# Autodesk Inventor assembly: Trunk
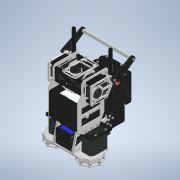
[picture p0: Inventor's stored thumbnail of the model, 180x180]
Saved by Autodesk Inventor 2020.4 (Build 244396000, 396)
## iProperties
Created: 2021-09-10
Part Number: Trunk
Document SubType Name: Assembly
Designer: Masato
Mass: 1616.91 g
Surface Area: 5782.28 cm^2
Volume: 882.028 cm^3
Density: 1.83317 g/cm^3
Author: Masato
## Documents named in this file (36)
- C:\Users\Masato\Documents\Inventor\CIT Brains_Inventor\OpenPlatform_ver3_0（ワッシャ変更）\UpperBody\Trunk\Trunk.iam
- C:\Users\Masato\Documents\Inventor\CIT Brains_Inventor\OpenPlatform_ver3_0（ワッシャ変更）\UpperBody\Trunk\Trunk_chest_horizontal_frame.ipt
- C:\Users\Masato\Documents\Inventor\CIT Brains_Inventor\OpenPlatform_ver3_0（ワッシャ変更）\UpperBody\Trunk\Trunk_chest_back_forth_frame.ipt
- C:\Users\Masato\Documents\Inventor\CIT Brains_Inventor\OpenPlatform_ver3_0（ワッシャ変更）\UpperBody\Trunk\Trunk_armpit_frame.ipt
- C:\Users\Masato\Documents\Inventor\CIT Brains_Inventor\OpenPlatform_ver3_0（ワッシャ変更）\UpperBody\Trunk\Trunk_abdomen_spacer.ipt
- C:\Users\Masato\Documents\Inventor\CIT Brains_Inventor\OpenPlatform_ver3_0（ワッシャ変更）\UpperBody\Trunk\Trunk_upper_flank_frame.ipt
- C:\Users\Masato\Documents\Inventor\CIT Brains_Inventor\OpenPlatform_ver3_0（ワッシャ変更）\UpperBody\Trunk\Trunk_shoulder_frame.ipt
- C:\Users\Masato\Documents\Inventor\CIT Brains_Inventor\OpenPlatform_ver3_0（ワッシャ変更）\UpperBody\Trunk\Trunk_handle_frame.ipt
- C:\Users\Masato\Documents\Inventor\CIT Brains_Inventor\OpenPlatform_ver3_0（ワッシャ変更）\UpperBody\Trunk\Trunk_chest_side_frame.ipt
- C:\Users\Masato\Documents\Inventor\CIT Brains_Inventor\OpenPlatform_ver3_0（ワッシャ変更）\Ready_Made\B3M11xx.ipt
- C:\Users\Masato\Documents\Inventor\CIT Brains_Inventor\OpenPlatform_ver3_0（ワッシャ変更）\Ready_Made\S3-07-3W.ipt
- C:\Users\Masato\Documents\Inventor\CIT Brains_Inventor\OpenPlatform_ver3_0（ワッシャ変更）\Ready_Made\ASU-375H.ipt
- C:\Users\Masato\Documents\Inventor\CIT Brains_Inventor\OpenPlatform_ver3_0（ワッシャ変更）\Ready_Made\B3M10xx.ipt
- C:\Users\Masato\Documents\Inventor\CIT Brains_Inventor\OpenPlatform_ver3_0（ワッシャ変更）\UpperBody\Cockpit\Cockpit.iam
- C:\Users\Masato\Documents\Inventor\CIT Brains_Inventor\OpenPlatform_ver3_0（ワッシャ変更）\UpperBody\Trunk\Trunk_shoulder_frame_MIR.ipt
- C:\Users\Masato\Documents\Inventor\CIT Brains_Inventor\OpenPlatform_ver3_0（ワッシャ変更）\UpperBody\Trunk\Trunk_lower_flank_frame.ipt
- C:\Users\Masato\Documents\Inventor\CIT Brains_Inventor\OpenPlatform_ver3_0（ワッシャ変更）\Ready_Made\Screw\SPNFL-BRN-M3-6.ipt
- C:\Users\Masato\Documents\Inventor\CIT Brains_Inventor\OpenPlatform_ver3_0（ワッシャ変更）\Ready_Made\Screw\M2_6-15.ipt
- C:\Users\Masato\Documents\Inventor\CIT Brains_Inventor\OpenPlatform_ver3_0（ワッシャ変更）\Ready_Made\Screw\M3-8.ipt
- C:\Users\Masato\Documents\Inventor\CIT Brains_Inventor\OpenPlatform_ver3_0（ワッシャ変更）\Ready_Made\Screw\M3-6.ipt
- C:\Users\Masato\Documents\Inventor\CIT Brains_Inventor\OpenPlatform_ver3_0（ワッシャ変更）\Ready_Made\Screw\M2_6-20.ipt
- C:\Users\Masato\Documents\Inventor\CIT Brains_Inventor\OpenPlatform_ver3_0（ワッシャ変更）\UpperBody\Trunk\Outer_support_stand.ipt
- C:\Users\Masato\Documents\Inventor\CIT Brains_Inventor\OpenPlatform_ver3_0（ワッシャ変更）\Ready_Made\BRU-307S.ipt
- C:\Users\Masato\Documents\Inventor\CIT Brains_Inventor\OpenPlatform_ver3_0（ワッシャ変更）\UpperBody\Trunk\Outer_flange.ipt
- C:\Users\Masato\Documents\Inventor\CIT Brains_Inventor\OpenPlatform_ver3_0（ワッシャ変更）\UpperBody\Trunk\Inner_flange.ipt
- C:\Users\Masato\Documents\Inventor\CIT Brains_Inventor\OpenPlatform_ver3_0（ワッシャ変更）\Ready_Made\CRBA02508WWC8P5\CRBA02508WWC8P5.ipt
- C:\Users\Masato\Documents\Inventor\CIT Brains_Inventor\OpenPlatform_ver3_0（ワッシャ変更）\UpperBody\Trunk\Inner_support_stand.ipt
- C:\Users\Masato\Documents\Inventor\CIT Brains_Inventor\OpenPlatform_ver3_0（ワッシャ変更）\UpperBody\Trunk\Trunk_lower_waisit_frame.ipt
- C:\Users\Masato\Documents\Inventor\CIT Brains_Inventor\OpenPlatform_ver3_0（ワッシャ変更）\Ready_Made\BRU-309S.ipt
- C:\Users\Masato\Documents\Inventor\CIT Brains_Inventor\OpenPlatform_ver3_0（ワッシャ変更）\UpperBody\Trunk\Trunk_upper_waist_frame.ipt
- C:\Users\Masato\Documents\Inventor\CIT Brains_Inventor\OpenPlatform_ver3_0（ワッシャ変更）\Ready_Made\UUW-0312-10BH.ipt
- C:\Users\Masato\Documents\Inventor\CIT Brains_Inventor\OpenPlatform_ver3_0（ワッシャ変更）\Ready_Made\Screw\M2_6-6.ipt
- C:\Users\Masato\Documents\Inventor\CIT Brains_Inventor\OpenPlatform_ver3_0（ワッシャ変更）\Ready_Made\ASU-309-6.ipt
- C:\Users\Masato\Documents\Inventor\CIT Brains_Inventor\OpenPlatform_ver3_0（ワッシャ変更）\Ready_Made\SLSBF7-134-M3-N3.ipt
- C:\Users\Masato\Documents\Inventor\CIT Brains_Inventor\OpenPlatform_ver3_0（ワッシャ変更）\Ready_Made\BRU-2608S.ipt
- C:\Users\Masato\Documents\Inventor\CIT Brains_Inventor\OpenPlatform_ver3_0（ワッシャ変更）\Ready_Made\SF319.ipt
## Components (214 placed, 35 different names)
1. Trunk_chest_horizontal_frame:1 — 挿入:172, 挿入:173, 挿入:174, 挿入:175, 挿入:177, 挿入:179, 挿入:255, 挿入:256, 挿入:261, 挿入:262, 挿入:347, 挿入:348, 挿入:463, 挿入:464
2. Trunk_chest_horizontal_frame:2 — 挿入:181, 挿入:182, 挿入:184, 挿入:185, 挿入:186, 挿入:187, 挿入:257, 挿入:258, 挿入:337, 挿入:338, 挿入:465, 挿入:466, 挿入:664, 挿入:665
3. Trunk_chest_back_forth_frame:1 — 挿入:115, 挿入:116, 挿入:117, 挿入:118, 挿入:172, 挿入:173, 挿入:181, 挿入:182
4. Trunk_chest_back_forth_frame:2 — 挿入:154, 挿入:155, 挿入:156, 挿入:157, 挿入:174, 挿入:175, 挿入:185, 挿入:187
5. Trunk_armpit_frame:1 — 挿入:111, 挿入:112, 挿入:555, 挿入:556
6. Trunk_armpit_frame:2 — 挿入:164, 挿入:165, 挿入:557, 挿入:558
7. Trunk_armpit_frame:3 — 挿入:229, 挿入:230, 挿入:577, 挿入:579
8. Trunk_armpit_frame:4 — 挿入:168, 挿入:169, 挿入:578, 挿入:580
9. Trunk_lower_flank_frame:1 — 挿入:420, 挿入:421, 挿入:426, 挿入:501, 挿入:502, 挿入:668, 挿入:669
10. Trunk_lower_flank_frame:2 — メイト:23, メイト:24, メイト:25, 挿入:418, 挿入:419, 挿入:499, 挿入:500, 挿入:666, 挿入:667
11. Trunk_abdomen_spacer:1 — フラッシュ:16, メイト:17, フラッシュ:18, フラッシュ:20, フラッシュ:21, メイト:22
12. Trunk_abdomen_spacer:2 — フラッシュ:16, メイト:17, フラッシュ:18, メイト:19
13. Trunk_abdomen_spacer:3 — フラッシュ:15, メイト:18, フラッシュ:17, フラッシュ:19, フラッシュ:20, フラッシュ:21, メイト:21, メイト:20
14. Trunk_abdomen_spacer:4 — フラッシュ:15, メイト:18, フラッシュ:17, メイト:25
15. Trunk_upper_flank_frame:1 — 挿入:101, 挿入:102, 挿入:103, 挿入:111, 挿入:112, 挿入:115, 挿入:116, 挿入:156, 挿入:157, 挿入:164, 挿入:165, フラッシュ:19, メイト:21, 挿入:208, 挿入:226, 挿入:245, 挿入:246, 挿入:247, 挿入:251, 挿入:252, 挿入:327, 挿入:328, 挿入:329, 挿入:330, 挿入:349, 挿入:350
16. Trunk_upper_flank_frame:2 — 挿入:104, 挿入:105, 挿入:106, 挿入:117, 挿入:118, 挿入:154, 挿入:155, 挿入:168, 挿入:169, メイト:22, 挿入:227, 挿入:229, 挿入:230, 挿入:248, 挿入:249, 挿入:250, 挿入:253, 挿入:254, 挿入:331, 挿入:332, 挿入:333, 挿入:334, 挿入:351, 挿入:352
17. Trunk_shoulder_frame:1 — 挿入:555, 挿入:556, 挿入:557, 挿入:558, 挿入:559, 挿入:560, 挿入:561, 挿入:562, 挿入:563, 挿入:564, 挿入:565, 挿入:566, 挿入:567, 挿入:568, 挿入:569, 挿入:570, 角度:48, 挿入:571, 角度:49, 挿入:572, 挿入:573, 挿入:574
18. Trunk_shoulder_frame_MIR:1 — 挿入:577, 挿入:578, 挿入:579, 挿入:580, 挿入:581, 挿入:582, 挿入:583, 挿入:584, 挿入:585, 挿入:586, 挿入:587, 挿入:588, 挿入:589, 挿入:590, 挿入:591, 挿入:592, 挿入:593, 挿入:594, 角度:50, 角度:51, 挿入:595, 挿入:596
19. Trunk_handle_frame:1 — 挿入:263, 挿入:264, 挿入:267, 挿入:575, 挿入:576, 角度:52, 挿入:599
20. Trunk_handle_frame:2 — 挿入:265, 挿入:266, 挿入:268, 挿入:597, 挿入:598
21. Trunk_chest_side_frame:1 — 挿入:467, 挿入:468, 挿入:469, 挿入:470, 挿入:471, 挿入:472, 挿入:473, 挿入:474
22. Trunk_chest_side_frame:2 — 挿入:475, 挿入:476, 挿入:477, 挿入:478, 挿入:479, 挿入:480, 挿入:481, 挿入:482
23. B3M11xx:1 — 角度:39, 挿入:391, 挿入:392, 挿入:422, 挿入:423, 挿入:424, 挿入:425, 挿入:483, 挿入:486, フラッシュ:23
24. B3M11xx:2 — 挿入:427, 挿入:428, 挿入:429, 挿入:484, 挿入:485, 挿入:529
25. B3M11xx:3 — 挿入:177, 挿入:179, 挿入:184, 挿入:186
26. B3M10xx:4 — 挿入:475, 挿入:476, 挿入:477, 挿入:478, 挿入:559, 挿入:560, 挿入:561, 挿入:562
27. B3M10xx:5 — 挿入:467, 挿入:468, 挿入:469, 挿入:470, 挿入:581, 挿入:582, 挿入:583, 挿入:584
28. ASU-375H:1 — フラッシュ:9, フラッシュ:10, フラッシュ:11, フラッシュ:12, 挿入:101, 挿入:104, メイト:19, メイト:20, メイト:23, メイト:24
29. ASU-375H:2 — フラッシュ:9, フラッシュ:11, 挿入:102, 挿入:105
30. ASU-375H:3 — フラッシュ:10, フラッシュ:12, 挿入:103, 挿入:106
31. Cockpit:1 [sub-assembly] — 挿入:208, 角度:39
32. SPNFL-BRN-M3-6:1 — 挿入:226
33. SPNFL-BRN-M3-6:2 — 挿入:227
34. M3-8:5 — 挿入:245
35. M3-8:6 — 挿入:246
36. M3-8:7 — 挿入:247
37. M3-8:8 — 挿入:248
38. M3-8:9 — 挿入:249
39. M3-8:10 — 挿入:250
40. M3-6:1 — 挿入:251
41. M3-6:2 — 挿入:252
42. M3-6:3 — 挿入:254
43. M3-6:4 — 挿入:253
44. M3-6:5 — 挿入:256
45. M3-6:6 — 挿入:255
46. M3-6:7 — 挿入:258
47. M3-6:8 — 挿入:257
48. M2_6-15:9 — 挿入:464
49. M2_6-15:10 — 挿入:463
50. M2_6-15:11 — 挿入:261
51. M2_6-15:12 — 挿入:262
52. M3-6:9 — 挿入:263
53. M3-6:10 — 挿入:264
54. M3-6:11 — 挿入:266
55. M3-6:12 — 挿入:265
56. M3-8:11 — 挿入:267
57. M3-8:12 — 挿入:268
58. M2_6-20:1 — 挿入:489
59. M2_6-20:2 — 挿入:490
60. M2_6-20:3 — 挿入:487
61. M2_6-20:4 — 挿入:488
62. M2_6-15:13 — 挿入:564
63. M2_6-15:14 — 挿入:563
64. M2_6-15:15 — 挿入:566
65. M2_6-15:16 — 挿入:565
66. M2_6-15:17 — 挿入:591
67. M2_6-15:18 — 挿入:592
68. M2_6-15:19 — 挿入:589
69. M2_6-15:20 — 挿入:590
70. M3-6:13 — 挿入:567
71. M3-6:14 — 挿入:568
72. M3-6:15 — 挿入:569
73. M3-6:16 — 挿入:570
74. M3-6:17 — 挿入:585
75. M3-6:18 — 挿入:586
76. M3-6:19 — 挿入:587
77. M3-6:20 — 挿入:588
78. M3-6:21 — 挿入:327
79. M3-6:22 — 挿入:328
80. M3-6:23 — 挿入:329
81. M3-6:24 — 挿入:330
82. M3-6:25 — 挿入:331
83. M3-6:26 — 挿入:332
84. M3-6:27 — 挿入:333
85. M3-6:28 — 挿入:334
86. M2_6-20:9 — 挿入:465
87. M2_6-20:10 — 挿入:466
88. M2_6-20:11 — 挿入:337
89. M2_6-20:12 — 挿入:338
90. M2_6-20:13 — 挿入:479
91. M2_6-20:14 — 挿入:482
92. M2_6-20:15 — 挿入:481
93. M2_6-20:16 — 挿入:480
94. M2_6-20:17 — 挿入:474
95. M2_6-20:18 — 挿入:472
96. M2_6-20:19 — 挿入:473
97. M2_6-20:20 — 挿入:471
98. M3-6:29 — 挿入:347
99. M3-6:30 — 挿入:348
100. M3-6:31 — 挿入:349
101. M3-6:32 — 挿入:350
102. M3-6:33 — 挿入:351
103. M3-6:34 — 挿入:352
104. Outer_support_stand:1 — 挿入:397, 挿入:600, 挿入:601, 挿入:602, 挿入:603, 挿入:604, 挿入:605, 挿入:606, 挿入:607, 挿入:608, 挿入:609
105. Inner_flange:1 — 挿入:391, 挿入:392, 挿入:652, 挿入:653, 挿入:654, 挿入:655
106. CRBA02508WWC8P5:1 — 挿入:397
107. Inner_support_stand:1 — 角度:53, 角度:54, 角度:55, 角度:56, 挿入:624, 挿入:625, 挿入:626, 挿入:627, 挿入:644, 挿入:645, 挿入:646, 挿入:647, 挿入:662, 挿入:663
108. S3-07-3W:9 — 角度:53, 挿入:625
109. S3-07-3W:10 — 角度:56, 挿入:626
110. S3-07-3W:11 — 角度:55, 挿入:627
111. S3-07-3W:12 — 角度:54, 挿入:624
112. Outer_flange:1 — 挿入:406, 挿入:407, 挿入:408, 挿入:409, 挿入:410, 挿入:411, 挿入:412, 挿入:413, 挿入:610, 挿入:611
113. M3-6:35 — 挿入:406
114. M3-6:36 — 挿入:407
115. M3-6:37 — 挿入:408
116. M3-6:38 — 挿入:409
117. M3-6:39 — 挿入:410
118. M3-6:40 — 挿入:411
119. M3-6:41 — 挿入:412
120. M3-6:42 — 挿入:413
121. Trunk_lower_waisit_frame:1 — 挿入:418, 挿入:419, 挿入:420, 挿入:421, 挿入:422, 挿入:423, 挿入:424, 挿入:425, 挿入:426, 挿入:427, 挿入:428, 挿入:429, 挿入:440, 挿入:441, 挿入:442, 挿入:443, 挿入:444, 挿入:445, 挿入:446, 挿入:447, 挿入:448, 挿入:449, 挿入:450, 挿入:451, フラッシュ:22, 挿入:600, 挿入:601, 挿入:612, 挿入:623
122. M2_6-15:21 — 挿入:441
123. M2_6-15:22 — 挿入:440
124. M2_6-15:23 — 挿入:442
125. M2_6-15:24 — 挿入:443
126. M2_6-15:25 — 挿入:444
127. M2_6-15:26 — 挿入:445
128. M2_6-15:27 — 挿入:446
129. M2_6-15:28 — 挿入:447
130. M3-8:13 — 挿入:448
131. M3-8:14 — 挿入:449
132. M3-8:15 — 挿入:450
133. M3-8:16 — 挿入:451
134. Trunk_upper_waist_frame:1 — 挿入:483, 挿入:484, 挿入:485, 挿入:486, 挿入:487, 挿入:488, 挿入:489, 挿入:490
135. BRU-307S:9 — 挿入:497, 挿入:503
136. BRU-307S:10 — 挿入:498, 挿入:504
137. BRU-307S:11 — 挿入:496, 挿入:506
138. BRU-307S:12 — 挿入:495, 挿入:505
139. UUW-0312-10BH:1 — 挿入:495, 挿入:507
140. UUW-0312-10BH:2 — 挿入:496, 挿入:508
141. UUW-0312-10BH:3 — 挿入:497, 挿入:509
142. UUW-0312-10BH:4 — 挿入:498, 挿入:510
143. UUW-0312-10BH:5 — 挿入:499, 挿入:505
144. UUW-0312-10BH:6 — 挿入:500, 挿入:506
145. UUW-0312-10BH:7 — 挿入:501, 挿入:503
146. UUW-0312-10BH:8 — 挿入:502, 挿入:504
147. M3-6:43 — 挿入:507
148. M3-6:44 — 挿入:508
149. M3-6:45 — 挿入:510
150. M3-6:46 — 挿入:509
151. Outer_support_stand:2 — 挿入:554, 挿入:612, 挿入:613, 挿入:614, 挿入:615, 挿入:616, 挿入:617, 挿入:618, 挿入:619, 挿入:620, 挿入:623
152. S3-07-3W:13 — 角度:59, 挿入:630
153. S3-07-3W:14 — 角度:58, 挿入:629
154. S3-07-3W:15 — 角度:60, 挿入:631
155. S3-07-3W:16 — 角度:57, 挿入:628
156. Inner_flange:2 — 挿入:529, 挿入:656, 挿入:657, 挿入:658, 挿入:659
157. Inner_support_stand:2 — 角度:57, 角度:58, 角度:59, 角度:60, 挿入:628, 挿入:629, 挿入:630, 挿入:631, 挿入:648, 挿入:649, 挿入:650, 挿入:651, 挿入:660, 挿入:661
158. Outer_flange:2 — 挿入:542, 挿入:543, 挿入:544, 挿入:545, 挿入:546, 挿入:547, 挿入:548, 挿入:549, 挿入:621, 挿入:622
159. M3-6:47 — 挿入:542
160. M3-6:48 — 挿入:543
161. M3-6:49 — 挿入:544
162. M3-6:50 — 挿入:545
163. M3-6:51 — 挿入:546
164. M3-6:52 — 挿入:547
165. M3-6:53 — 挿入:548
166. M3-6:54 — 挿入:549
167. CRBA02508WWC8P5:2 — 挿入:554
168. ASU-309-6:1 — 角度:48, 挿入:571, 挿入:576
169. ASU-309-6:2 — 角度:49, 挿入:572, 挿入:575
170. M3-6:55 — 挿入:573
171. M3-6:56 — 挿入:574
172. M3-6:57 — 挿入:593
173. M3-6:58 — 挿入:594
174. ASU-309-6:3 — 角度:50, 挿入:595, 挿入:597
175. ASU-309-6:4 — 角度:51, 挿入:596, 挿入:598
176. SLSBF7-134-M3-N3:1 — 角度:52, 挿入:599
177. BRU-309S:17 — 挿入:602, 挿入:610
178. BRU-309S:18 — 挿入:603
179. BRU-309S:19 — 挿入:604
180. BRU-309S:20 — 挿入:605
181. BRU-309S:21 — 挿入:606, 挿入:611
182. BRU-309S:22 — 挿入:607
183. BRU-309S:23 — 挿入:608
184. BRU-309S:24 — 挿入:609
185. BRU-309S:25 — 挿入:617
186. BRU-309S:26 — 挿入:616
187. BRU-309S:27 — 挿入:615
188. BRU-309S:28 — 挿入:613, 挿入:621
189. BRU-309S:29 — 挿入:614
190. BRU-309S:30 — 挿入:618
191. BRU-309S:31 — 挿入:619
192. BRU-309S:32 — 挿入:620, 挿入:622
193. M2_6-6:1 — 挿入:644
194. M2_6-6:2 — 挿入:645
195. M2_6-6:3 — 挿入:646
196. M2_6-6:4 — 挿入:647
197. M2_6-6:5 — 挿入:651
198. M2_6-6:6 — 挿入:650
199. M2_6-6:7 — 挿入:649
200. M2_6-6:8 — 挿入:648
201. BRU-2608S:1 — 挿入:653, 挿入:662
202. BRU-2608S:2 — 挿入:654, 挿入:663
203. BRU-2608S:3 — 挿入:655
204. BRU-2608S:4 — 挿入:652
205. BRU-2608S:5 — 挿入:657, 挿入:660
206. BRU-2608S:6 — 挿入:656
207. BRU-2608S:7 — 挿入:658
208. BRU-2608S:8 — 挿入:659, 挿入:661
209. M3-6:59 — 挿入:664
210. M3-6:60 — 挿入:665
211. SF319:1 — 挿入:666
212. SF319:2 — 挿入:667
213. SF319:3 — 挿入:668
214. SF319:4 — 挿入:669
## Relationships (303: Insert 267, Angle 14, Flush 13, Mate 9)
- フラッシュ:9 [Flush]: ASU-375H:1 ↔ ASU-375H:2
- フラッシュ:10 [Flush]: ASU-375H:1 ↔ ASU-375H:3
- フラッシュ:11 [Flush]: ASU-375H:1 ↔ ASU-375H:2
- フラッシュ:12 [Flush]: ASU-375H:1 ↔ ASU-375H:3
- 挿入:101 [Insert]: Trunk_upper_flank_frame:1 ↔ ASU-375H:1
- 挿入:102 [Insert]: Trunk_upper_flank_frame:1 ↔ ASU-375H:2
- 挿入:103 [Insert]: Trunk_upper_flank_frame:1 ↔ ASU-375H:3
- 挿入:104 [Insert]: Trunk_upper_flank_frame:2 ↔ ASU-375H:1
- 挿入:105 [Insert]: Trunk_upper_flank_frame:2 ↔ ASU-375H:2
- 挿入:106 [Insert]: Trunk_upper_flank_frame:2 ↔ ASU-375H:3
- 挿入:111 [Insert]: Trunk_armpit_frame:1 ↔ Trunk_upper_flank_frame:1
- 挿入:112 [Insert]: Trunk_armpit_frame:1 ↔ Trunk_upper_flank_frame:1
- 挿入:115 [Insert]: Trunk_chest_back_forth_frame:1 ↔ Trunk_upper_flank_frame:1
- 挿入:116 [Insert]: Trunk_chest_back_forth_frame:1 ↔ Trunk_upper_flank_frame:1
- 挿入:117 [Insert]: Trunk_chest_back_forth_frame:1 ↔ Trunk_upper_flank_frame:2
- 挿入:118 [Insert]: Trunk_chest_back_forth_frame:1 ↔ Trunk_upper_flank_frame:2
- 挿入:154 [Insert]: Trunk_chest_back_forth_frame:2 ↔ Trunk_upper_flank_frame:2
- 挿入:155 [Insert]: Trunk_chest_back_forth_frame:2 ↔ Trunk_upper_flank_frame:2
- 挿入:156 [Insert]: Trunk_chest_back_forth_frame:2 ↔ Trunk_upper_flank_frame:1
- 挿入:157 [Insert]: Trunk_chest_back_forth_frame:2 ↔ Trunk_upper_flank_frame:1
- 挿入:164 [Insert]: Trunk_armpit_frame:2 ↔ Trunk_upper_flank_frame:1
- 挿入:165 [Insert]: Trunk_armpit_frame:2 ↔ Trunk_upper_flank_frame:1
- 挿入:168 [Insert]: Trunk_armpit_frame:4 ↔ Trunk_upper_flank_frame:2
- 挿入:169 [Insert]: Trunk_armpit_frame:4 ↔ Trunk_upper_flank_frame:2
- 挿入:172 [Insert]: Trunk_chest_horizontal_frame:1 ↔ Trunk_chest_back_forth_frame:1
- 挿入:173 [Insert]: Trunk_chest_horizontal_frame:1 ↔ Trunk_chest_back_forth_frame:1
- 挿入:174 [Insert]: Trunk_chest_horizontal_frame:1 ↔ Trunk_chest_back_forth_frame:2
- 挿入:175 [Insert]: Trunk_chest_horizontal_frame:1 ↔ Trunk_chest_back_forth_frame:2
- 挿入:177 [Insert]: Trunk_chest_horizontal_frame:1 ↔ B3M11xx:3
- 挿入:179 [Insert]: Trunk_chest_horizontal_frame:1 ↔ B3M11xx:3
- 挿入:181 [Insert]: Trunk_chest_horizontal_frame:2 ↔ Trunk_chest_back_forth_frame:1
- 挿入:182 [Insert]: Trunk_chest_horizontal_frame:2 ↔ Trunk_chest_back_forth_frame:1
- 挿入:184 [Insert]: Trunk_chest_horizontal_frame:2 ↔ B3M11xx:3
- 挿入:185 [Insert]: Trunk_chest_horizontal_frame:2 ↔ Trunk_chest_back_forth_frame:2
- 挿入:186 [Insert]: Trunk_chest_horizontal_frame:2 ↔ B3M11xx:3
- 挿入:187 [Insert]: Trunk_chest_horizontal_frame:2 ↔ Trunk_chest_back_forth_frame:2
- フラッシュ:15 [Flush]: Trunk_abdomen_spacer:3 ↔ Trunk_abdomen_spacer:4
- フラッシュ:16 [Flush]: Trunk_abdomen_spacer:1 ↔ Trunk_abdomen_spacer:2
- メイト:17 [Mate]: Trunk_abdomen_spacer:1 ↔ Trunk_abdomen_spacer:2
- メイト:18 [Mate]: Trunk_abdomen_spacer:3 ↔ Trunk_abdomen_spacer:4
- フラッシュ:17 [Flush]: Trunk_abdomen_spacer:3 ↔ Trunk_abdomen_spacer:4
- フラッシュ:18 [Flush]: Trunk_abdomen_spacer:1 ↔ Trunk_abdomen_spacer:2
- フラッシュ:19 [Flush]: Trunk_abdomen_spacer:3 ↔ Trunk_upper_flank_frame:1
- フラッシュ:20 [Flush]: Trunk_abdomen_spacer:1 ↔ Trunk_abdomen_spacer:3
- メイト:19 [Mate] (0.01 mm): Trunk_abdomen_spacer:2 ↔ ASU-375H:1
- メイト:20 [Mate] (0.01 mm): Trunk_abdomen_spacer:3 ↔ ASU-375H:1
- フラッシュ:21 [Flush]: Trunk_abdomen_spacer:1 ↔ Trunk_abdomen_spacer:3
- メイト:21 [Mate]: Trunk_abdomen_spacer:3 ↔ Trunk_upper_flank_frame:1
- メイト:22 [Mate]: Trunk_abdomen_spacer:1 ↔ Trunk_upper_flank_frame:2
- メイト:23 [Mate] (0.01 mm): Trunk_lower_flank_frame:2 ↔ ASU-375H:1
- メイト:24 [Mate] (0.01 mm): Trunk_lower_flank_frame:2 ↔ ASU-375H:1
- メイト:25 [Mate]: Trunk_lower_flank_frame:2 ↔ Trunk_abdomen_spacer:4
- 挿入:208 [Insert] (0.25 mm): Trunk_upper_flank_frame:1 ↔ Cockpit:1
- 角度:39 [Angle] (0 deg): B3M11xx:1 ↔ Cockpit:1
- 挿入:226 [Insert]: Trunk_upper_flank_frame:1 ↔ SPNFL-BRN-M3-6:1
- 挿入:227 [Insert]: Trunk_upper_flank_frame:2 ↔ SPNFL-BRN-M3-6:2
- 挿入:229 [Insert]: Trunk_armpit_frame:3 ↔ Trunk_upper_flank_frame:2
- 挿入:230 [Insert]: Trunk_armpit_frame:3 ↔ Trunk_upper_flank_frame:2
- 挿入:245 [Insert]: Trunk_upper_flank_frame:1 ↔ M3-8:5
- 挿入:246 [Insert]: Trunk_upper_flank_frame:1 ↔ M3-8:6
- 挿入:247 [Insert]: Trunk_upper_flank_frame:1 ↔ M3-8:7
- 挿入:248 [Insert]: Trunk_upper_flank_frame:2 ↔ M3-8:8
- 挿入:249 [Insert]: Trunk_upper_flank_frame:2 ↔ M3-8:9
- 挿入:250 [Insert]: Trunk_upper_flank_frame:2 ↔ M3-8:10
- 挿入:251 [Insert]: Trunk_upper_flank_frame:1 ↔ M3-6:1
- 挿入:252 [Insert]: Trunk_upper_flank_frame:1 ↔ M3-6:2
- 挿入:253 [Insert]: Trunk_upper_flank_frame:2 ↔ M3-6:4
- 挿入:254 [Insert]: Trunk_upper_flank_frame:2 ↔ M3-6:3
- 挿入:255 [Insert]: Trunk_chest_horizontal_frame:1 ↔ M3-6:6
- 挿入:256 [Insert]: Trunk_chest_horizontal_frame:1 ↔ M3-6:5
- 挿入:257 [Insert]: Trunk_chest_horizontal_frame:2 ↔ M3-6:8
- 挿入:258 [Insert]: Trunk_chest_horizontal_frame:2 ↔ M3-6:7
- 挿入:261 [Insert]: Trunk_chest_horizontal_frame:1 ↔ M2_6-15:11
- 挿入:262 [Insert]: Trunk_chest_horizontal_frame:1 ↔ M2_6-15:12
- 挿入:263 [Insert]: Trunk_handle_frame:1 ↔ M3-6:9
- 挿入:264 [Insert]: Trunk_handle_frame:1 ↔ M3-6:10
- 挿入:265 [Insert]: Trunk_handle_frame:2 ↔ M3-6:12
- 挿入:266 [Insert]: Trunk_handle_frame:2 ↔ M3-6:11
- 挿入:267 [Insert]: Trunk_handle_frame:1 ↔ M3-8:11
- 挿入:268 [Insert]: Trunk_handle_frame:2 ↔ M3-8:12
- 挿入:327 [Insert]: Trunk_upper_flank_frame:1 ↔ M3-6:21
- 挿入:328 [Insert]: Trunk_upper_flank_frame:1 ↔ M3-6:22
- 挿入:329 [Insert]: Trunk_upper_flank_frame:1 ↔ M3-6:23
- 挿入:330 [Insert]: Trunk_upper_flank_frame:1 ↔ M3-6:24
- 挿入:331 [Insert]: Trunk_upper_flank_frame:2 ↔ M3-6:25
- 挿入:332 [Insert]: Trunk_upper_flank_frame:2 ↔ M3-6:26
- 挿入:333 [Insert]: Trunk_upper_flank_frame:2 ↔ M3-6:27
- 挿入:334 [Insert]: Trunk_upper_flank_frame:2 ↔ M3-6:28
- 挿入:337 [Insert]: Trunk_chest_horizontal_frame:2 ↔ M2_6-20:11
- 挿入:338 [Insert]: Trunk_chest_horizontal_frame:2 ↔ M2_6-20:12
- 挿入:347 [Insert]: Trunk_chest_horizontal_frame:1 ↔ M3-6:29
- 挿入:348 [Insert]: Trunk_chest_horizontal_frame:1 ↔ M3-6:30
- 挿入:349 [Insert]: Trunk_upper_flank_frame:1 ↔ M3-6:31
- 挿入:350 [Insert]: Trunk_upper_flank_frame:1 ↔ M3-6:32
- 挿入:351 [Insert]: Trunk_upper_flank_frame:2 ↔ M3-6:33
- 挿入:352 [Insert]: Trunk_upper_flank_frame:2 ↔ M3-6:34
- 挿入:391 [Insert]: B3M11xx:1 ↔ Inner_flange:1
- 挿入:392 [Insert]: B3M11xx:1 ↔ Inner_flange:1
- 挿入:397 [Insert]: Outer_support_stand:1 ↔ CRBA02508WWC8P5:1
- 挿入:406 [Insert]: Outer_flange:1 ↔ M3-6:35
- 挿入:407 [Insert]: Outer_flange:1 ↔ M3-6:36
- 挿入:408 [Insert]: Outer_flange:1 ↔ M3-6:37
- 挿入:409 [Insert]: Outer_flange:1 ↔ M3-6:38
- 挿入:410 [Insert]: Outer_flange:1 ↔ M3-6:39
- 挿入:411 [Insert]: Outer_flange:1 ↔ M3-6:40
- 挿入:412 [Insert]: Outer_flange:1 ↔ M3-6:41
- 挿入:413 [Insert]: Outer_flange:1 ↔ M3-6:42
- 挿入:418 [Insert]: Trunk_lower_flank_frame:2 ↔ Trunk_lower_waisit_frame:1
- 挿入:419 [Insert]: Trunk_lower_flank_frame:2 ↔ Trunk_lower_waisit_frame:1
- 挿入:420 [Insert]: Trunk_lower_flank_frame:1 ↔ Trunk_lower_waisit_frame:1
- 挿入:421 [Insert]: Trunk_lower_flank_frame:1 ↔ Trunk_lower_waisit_frame:1
- 挿入:422 [Insert]: B3M11xx:1 ↔ Trunk_lower_waisit_frame:1
- 挿入:423 [Insert]: B3M11xx:1 ↔ Trunk_lower_waisit_frame:1
- 挿入:424 [Insert]: B3M11xx:1 ↔ Trunk_lower_waisit_frame:1
- 挿入:425 [Insert]: B3M11xx:1 ↔ Trunk_lower_waisit_frame:1
- 挿入:426 [Insert]: Trunk_lower_flank_frame:1 ↔ Trunk_lower_waisit_frame:1
- 挿入:427 [Insert]: B3M11xx:2 ↔ Trunk_lower_waisit_frame:1
- 挿入:428 [Insert]: B3M11xx:2 ↔ Trunk_lower_waisit_frame:1
- 挿入:429 [Insert]: B3M11xx:2 ↔ Trunk_lower_waisit_frame:1
- 挿入:440 [Insert]: Trunk_lower_waisit_frame:1 ↔ M2_6-15:22
- 挿入:441 [Insert]: Trunk_lower_waisit_frame:1 ↔ M2_6-15:21
- 挿入:442 [Insert]: Trunk_lower_waisit_frame:1 ↔ M2_6-15:23
- 挿入:443 [Insert]: Trunk_lower_waisit_frame:1 ↔ M2_6-15:24
- 挿入:444 [Insert]: Trunk_lower_waisit_frame:1 ↔ M2_6-15:25
- 挿入:445 [Insert]: Trunk_lower_waisit_frame:1 ↔ M2_6-15:26
- 挿入:446 [Insert]: Trunk_lower_waisit_frame:1 ↔ M2_6-15:27
- 挿入:447 [Insert]: Trunk_lower_waisit_frame:1 ↔ M2_6-15:28
- 挿入:448 [Insert]: Trunk_lower_waisit_frame:1 ↔ M3-8:13
- 挿入:449 [Insert]: Trunk_lower_waisit_frame:1 ↔ M3-8:14
- 挿入:450 [Insert]: Trunk_lower_waisit_frame:1 ↔ M3-8:15
- 挿入:451 [Insert]: Trunk_lower_waisit_frame:1 ↔ M3-8:16
- フラッシュ:22 [Flush]: Trunk_lower_waisit_frame:1
- 挿入:463 [Insert]: Trunk_chest_horizontal_frame:1 ↔ M2_6-15:10
- 挿入:464 [Insert]: Trunk_chest_horizontal_frame:1 ↔ M2_6-15:9
- 挿入:465 [Insert]: Trunk_chest_horizontal_frame:2 ↔ M2_6-20:9
- 挿入:466 [Insert]: Trunk_chest_horizontal_frame:2 ↔ M2_6-20:10
- 挿入:467 [Insert]: Trunk_chest_side_frame:1 ↔ B3M10xx:5
- 挿入:468 [Insert]: Trunk_chest_side_frame:1 ↔ B3M10xx:5
- 挿入:469 [Insert]: Trunk_chest_side_frame:1 ↔ B3M10xx:5
- 挿入:470 [Insert]: Trunk_chest_side_frame:1 ↔ B3M10xx:5
- 挿入:471 [Insert]: Trunk_chest_side_frame:1 ↔ M2_6-20:20
- 挿入:472 [Insert]: Trunk_chest_side_frame:1 ↔ M2_6-20:18
- 挿入:473 [Insert]: Trunk_chest_side_frame:1 ↔ M2_6-20:19
- 挿入:474 [Insert]: Trunk_chest_side_frame:1 ↔ M2_6-20:17
- 挿入:475 [Insert]: Trunk_chest_side_frame:2 ↔ B3M10xx:4
- 挿入:476 [Insert]: Trunk_chest_side_frame:2 ↔ B3M10xx:4
- 挿入:477 [Insert]: Trunk_chest_side_frame:2 ↔ B3M10xx:4
- 挿入:478 [Insert]: Trunk_chest_side_frame:2 ↔ B3M10xx:4
- 挿入:479 [Insert]: Trunk_chest_side_frame:2 ↔ M2_6-20:13
- 挿入:480 [Insert]: Trunk_chest_side_frame:2 ↔ M2_6-20:16
- 挿入:481 [Insert]: Trunk_chest_side_frame:2 ↔ M2_6-20:15
- 挿入:482 [Insert]: Trunk_chest_side_frame:2 ↔ M2_6-20:14
- 挿入:483 [Insert]: B3M11xx:1 ↔ Trunk_upper_waist_frame:1
- 挿入:484 [Insert]: B3M11xx:2 ↔ Trunk_upper_waist_frame:1
- 挿入:485 [Insert]: B3M11xx:2 ↔ Trunk_upper_waist_frame:1
- 挿入:486 [Insert]: B3M11xx:1 ↔ Trunk_upper_waist_frame:1
- 挿入:487 [Insert]: M2_6-20:3 ↔ Trunk_upper_waist_frame:1
- 挿入:488 [Insert]: M2_6-20:4 ↔ Trunk_upper_waist_frame:1
- 挿入:489 [Insert]: M2_6-20:1 ↔ Trunk_upper_waist_frame:1
- 挿入:490 [Insert]: M2_6-20:2 ↔ Trunk_upper_waist_frame:1
- 挿入:495 [Insert]: BRU-307S:12 ↔ UUW-0312-10BH:1
- 挿入:496 [Insert]: BRU-307S:11 ↔ UUW-0312-10BH:2
- 挿入:497 [Insert]: BRU-307S:9 ↔ UUW-0312-10BH:3
- 挿入:498 [Insert]: BRU-307S:10 ↔ UUW-0312-10BH:4
- 挿入:499 [Insert]: Trunk_lower_flank_frame:2 ↔ UUW-0312-10BH:5
- 挿入:500 [Insert]: Trunk_lower_flank_frame:2 ↔ UUW-0312-10BH:6
- 挿入:501 [Insert]: Trunk_lower_flank_frame:1 ↔ UUW-0312-10BH:7
- 挿入:502 [Insert]: Trunk_lower_flank_frame:1 ↔ UUW-0312-10BH:8
- 挿入:503 [Insert]: BRU-307S:9 ↔ UUW-0312-10BH:7
- 挿入:504 [Insert]: BRU-307S:10 ↔ UUW-0312-10BH:8
- 挿入:505 [Insert]: BRU-307S:12 ↔ UUW-0312-10BH:5
- 挿入:506 [Insert]: BRU-307S:11 ↔ UUW-0312-10BH:6
- 挿入:507 [Insert]: UUW-0312-10BH:1 ↔ M3-6:43
- 挿入:508 [Insert]: UUW-0312-10BH:2 ↔ M3-6:44
- 挿入:509 [Insert]: UUW-0312-10BH:3 ↔ M3-6:46
- 挿入:510 [Insert]: UUW-0312-10BH:4 ↔ M3-6:45
- 挿入:529 [Insert]: B3M11xx:2 ↔ Inner_flange:2
- 挿入:542 [Insert]: Outer_flange:2 ↔ M3-6:47
- 挿入:543 [Insert]: Outer_flange:2 ↔ M3-6:48
- 挿入:544 [Insert]: Outer_flange:2 ↔ M3-6:49
- 挿入:545 [Insert]: Outer_flange:2 ↔ M3-6:50
- 挿入:546 [Insert]: Outer_flange:2 ↔ M3-6:51
- 挿入:547 [Insert]: Outer_flange:2 ↔ M3-6:52
- 挿入:548 [Insert]: Outer_flange:2 ↔ M3-6:53
- 挿入:549 [Insert]: Outer_flange:2 ↔ M3-6:54
- 挿入:554 [Insert]: Outer_support_stand:2 ↔ CRBA02508WWC8P5:2
- 挿入:555 [Insert]: Trunk_armpit_frame:1 ↔ Trunk_shoulder_frame:1
- 挿入:556 [Insert]: Trunk_armpit_frame:1 ↔ Trunk_shoulder_frame:1
- 挿入:557 [Insert]: Trunk_armpit_frame:2 ↔ Trunk_shoulder_frame:1
- 挿入:558 [Insert]: Trunk_armpit_frame:2 ↔ Trunk_shoulder_frame:1
- 挿入:559 [Insert]: Trunk_shoulder_frame:1 ↔ B3M10xx:4
- 挿入:560 [Insert]: Trunk_shoulder_frame:1 ↔ B3M10xx:4
- 挿入:561 [Insert]: Trunk_shoulder_frame:1 ↔ B3M10xx:4
- 挿入:562 [Insert]: Trunk_shoulder_frame:1 ↔ B3M10xx:4
- 挿入:563 [Insert]: Trunk_shoulder_frame:1 ↔ M2_6-15:14
- 挿入:564 [Insert]: Trunk_shoulder_frame:1 ↔ M2_6-15:13
- 挿入:565 [Insert]: Trunk_shoulder_frame:1 ↔ M2_6-15:16
- 挿入:566 [Insert]: Trunk_shoulder_frame:1 ↔ M2_6-15:15
- 挿入:567 [Insert]: Trunk_shoulder_frame:1 ↔ M3-6:13
- 挿入:568 [Insert]: Trunk_shoulder_frame:1 ↔ M3-6:14
- 挿入:569 [Insert]: Trunk_shoulder_frame:1 ↔ M3-6:15
- 挿入:570 [Insert]: Trunk_shoulder_frame:1 ↔ M3-6:16
- 角度:48 [Angle] (0 deg): Trunk_shoulder_frame:1 ↔ ASU-309-6:1
- 挿入:571 [Insert]: Trunk_shoulder_frame:1 ↔ ASU-309-6:1
- 角度:49 [Angle] (0 deg): Trunk_shoulder_frame:1 ↔ ASU-309-6:2
- 挿入:572 [Insert]: Trunk_shoulder_frame:1 ↔ ASU-309-6:2
- 挿入:573 [Insert]: Trunk_shoulder_frame:1 ↔ M3-6:55
- 挿入:574 [Insert]: Trunk_shoulder_frame:1 ↔ M3-6:56
- 挿入:575 [Insert]: Trunk_handle_frame:1 ↔ ASU-309-6:2
- 挿入:576 [Insert]: Trunk_handle_frame:1 ↔ ASU-309-6:1
- 挿入:577 [Insert]: Trunk_armpit_frame:3 ↔ Trunk_shoulder_frame_MIR:1
- 挿入:578 [Insert]: Trunk_armpit_frame:4 ↔ Trunk_shoulder_frame_MIR:1
- 挿入:579 [Insert]: Trunk_armpit_frame:3 ↔ Trunk_shoulder_frame_MIR:1
- 挿入:580 [Insert]: Trunk_armpit_frame:4 ↔ Trunk_shoulder_frame_MIR:1
- 挿入:581 [Insert]: Trunk_shoulder_frame_MIR:1 ↔ B3M10xx:5
- 挿入:582 [Insert]: Trunk_shoulder_frame_MIR:1 ↔ B3M10xx:5
- 挿入:583 [Insert]: Trunk_shoulder_frame_MIR:1 ↔ B3M10xx:5
- 挿入:584 [Insert]: Trunk_shoulder_frame_MIR:1 ↔ B3M10xx:5
- 挿入:585 [Insert]: Trunk_shoulder_frame_MIR:1 ↔ M3-6:17
- 挿入:586 [Insert]: Trunk_shoulder_frame_MIR:1 ↔ M3-6:18
- 挿入:587 [Insert]: Trunk_shoulder_frame_MIR:1 ↔ M3-6:19
- 挿入:588 [Insert]: Trunk_shoulder_frame_MIR:1 ↔ M3-6:20
- 挿入:589 [Insert]: Trunk_shoulder_frame_MIR:1 ↔ M2_6-15:19
- 挿入:590 [Insert]: Trunk_shoulder_frame_MIR:1 ↔ M2_6-15:20
- 挿入:591 [Insert]: Trunk_shoulder_frame_MIR:1 ↔ M2_6-15:17
- 挿入:592 [Insert]: Trunk_shoulder_frame_MIR:1 ↔ M2_6-15:18
- 挿入:593 [Insert]: Trunk_shoulder_frame_MIR:1 ↔ M3-6:57
- 挿入:594 [Insert]: Trunk_shoulder_frame_MIR:1 ↔ M3-6:58
- 角度:50 [Angle] (0 deg): Trunk_shoulder_frame_MIR:1 ↔ ASU-309-6:3
- 角度:51 [Angle] (0 deg): Trunk_shoulder_frame_MIR:1 ↔ ASU-309-6:4
- 挿入:595 [Insert]: Trunk_shoulder_frame_MIR:1 ↔ ASU-309-6:3
- 挿入:596 [Insert]: Trunk_shoulder_frame_MIR:1 ↔ ASU-309-6:4
- 挿入:597 [Insert]: Trunk_handle_frame:2 ↔ ASU-309-6:3
- 挿入:598 [Insert]: Trunk_handle_frame:2 ↔ ASU-309-6:4
- 角度:52 [Angle] (0 deg): Trunk_handle_frame:1 ↔ SLSBF7-134-M3-N3:1
- 挿入:599 [Insert]: Trunk_handle_frame:1 ↔ SLSBF7-134-M3-N3:1
- フラッシュ:23 [Flush] (-60 mm): B3M11xx:1
- 挿入:600 [Insert]: Outer_support_stand:1 ↔ Trunk_lower_waisit_frame:1
- 挿入:601 [Insert]: Outer_support_stand:1 ↔ Trunk_lower_waisit_frame:1
- 挿入:602 [Insert]: Outer_support_stand:1 ↔ BRU-309S:17
- 挿入:603 [Insert]: Outer_support_stand:1 ↔ BRU-309S:18
- 挿入:604 [Insert]: Outer_support_stand:1 ↔ BRU-309S:19
- 挿入:605 [Insert]: Outer_support_stand:1 ↔ BRU-309S:20
- 挿入:606 [Insert]: Outer_support_stand:1 ↔ BRU-309S:21
- 挿入:607 [Insert]: Outer_support_stand:1 ↔ BRU-309S:22
- 挿入:608 [Insert]: Outer_support_stand:1 ↔ BRU-309S:23
- 挿入:609 [Insert]: Outer_support_stand:1 ↔ BRU-309S:24
- 挿入:610 [Insert]: Outer_flange:1 ↔ BRU-309S:17
- 挿入:611 [Insert]: Outer_flange:1 ↔ BRU-309S:21
- 挿入:612 [Insert]: Trunk_lower_waisit_frame:1 ↔ Outer_support_stand:2
- 挿入:613 [Insert]: Outer_support_stand:2 ↔ BRU-309S:28
- 挿入:614 [Insert]: Outer_support_stand:2 ↔ BRU-309S:29
- 挿入:615 [Insert]: Outer_support_stand:2 ↔ BRU-309S:27
- 挿入:616 [Insert]: Outer_support_stand:2 ↔ BRU-309S:26
- 挿入:617 [Insert]: Outer_support_stand:2 ↔ BRU-309S:25
- 挿入:618 [Insert]: Outer_support_stand:2 ↔ BRU-309S:30
- 挿入:619 [Insert]: Outer_support_stand:2 ↔ BRU-309S:31
- 挿入:620 [Insert]: Outer_support_stand:2 ↔ BRU-309S:32
- 挿入:621 [Insert]: Outer_flange:2 ↔ BRU-309S:28
- 挿入:622 [Insert]: Outer_flange:2 ↔ BRU-309S:32
- 挿入:623 [Insert]: Trunk_lower_waisit_frame:1 ↔ Outer_support_stand:2
- 角度:53 [Angle] (0 deg): Inner_support_stand:1 ↔ S3-07-3W:9
- 角度:54 [Angle] (0 deg): Inner_support_stand:1 ↔ S3-07-3W:12
- 角度:55 [Angle] (0 deg): Inner_support_stand:1 ↔ S3-07-3W:11
- 角度:56 [Angle] (0 deg): Inner_support_stand:1 ↔ S3-07-3W:10
- 挿入:624 [Insert]: Inner_support_stand:1 ↔ S3-07-3W:12
- 挿入:625 [Insert]: Inner_support_stand:1 ↔ S3-07-3W:9
- 挿入:626 [Insert]: Inner_support_stand:1 ↔ S3-07-3W:10
- 挿入:627 [Insert]: Inner_support_stand:1 ↔ S3-07-3W:11
- 角度:57 [Angle] (0 deg): S3-07-3W:16 ↔ Inner_support_stand:2
- 角度:58 [Angle] (0 deg): S3-07-3W:14 ↔ Inner_support_stand:2
- 角度:59 [Angle] (0 deg): S3-07-3W:13 ↔ Inner_support_stand:2
- 角度:60 [Angle] (0 deg): S3-07-3W:15 ↔ Inner_support_stand:2
- 挿入:628 [Insert]: S3-07-3W:16 ↔ Inner_support_stand:2
- 挿入:629 [Insert]: S3-07-3W:14 ↔ Inner_support_stand:2
- 挿入:630 [Insert]: S3-07-3W:13 ↔ Inner_support_stand:2
- 挿入:631 [Insert]: S3-07-3W:15 ↔ Inner_support_stand:2
- 挿入:644 [Insert]: Inner_support_stand:1 ↔ M2_6-6:1
- 挿入:645 [Insert]: Inner_support_stand:1 ↔ M2_6-6:2
- 挿入:646 [Insert]: Inner_support_stand:1 ↔ M2_6-6:3
- 挿入:647 [Insert]: Inner_support_stand:1 ↔ M2_6-6:4
- 挿入:648 [Insert]: Inner_support_stand:2 ↔ M2_6-6:8
- 挿入:649 [Insert]: Inner_support_stand:2 ↔ M2_6-6:7
- 挿入:650 [Insert]: Inner_support_stand:2 ↔ M2_6-6:6
- 挿入:651 [Insert]: Inner_support_stand:2 ↔ M2_6-6:5
- 挿入:652 [Insert]: Inner_flange:1 ↔ BRU-2608S:4
- 挿入:653 [Insert]: Inner_flange:1 ↔ BRU-2608S:1
- 挿入:654 [Insert]: Inner_flange:1 ↔ BRU-2608S:2
- 挿入:655 [Insert]: Inner_flange:1 ↔ BRU-2608S:3
- 挿入:656 [Insert]: Inner_flange:2 ↔ BRU-2608S:6
- 挿入:657 [Insert]: Inner_flange:2 ↔ BRU-2608S:5
- 挿入:658 [Insert]: Inner_flange:2 ↔ BRU-2608S:7
- 挿入:659 [Insert]: Inner_flange:2 ↔ BRU-2608S:8
- 挿入:660 [Insert]: Inner_support_stand:2 ↔ BRU-2608S:5
- 挿入:661 [Insert]: Inner_support_stand:2 ↔ BRU-2608S:8
- 挿入:662 [Insert]: Inner_support_stand:1 ↔ BRU-2608S:1
- 挿入:663 [Insert]: Inner_support_stand:1 ↔ BRU-2608S:2
- 挿入:664 [Insert]: Trunk_chest_horizontal_frame:2 ↔ M3-6:59
- 挿入:665 [Insert]: Trunk_chest_horizontal_frame:2 ↔ M3-6:60
- 挿入:666 [Insert]: Trunk_lower_flank_frame:2 ↔ SF319:1
- 挿入:667 [Insert]: Trunk_lower_flank_frame:2 ↔ SF319:2
- 挿入:668 [Insert]: Trunk_lower_flank_frame:1 ↔ SF319:3
- 挿入:669 [Insert]: Trunk_lower_flank_frame:1 ↔ SF319:4
